# Autodesk Inventor assembly: Estructura Lámina
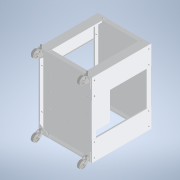
[picture p0: Inventor's stored thumbnail of the model, 180x180]
Saved by Autodesk Inventor 2021 (Build 250183000, 183)
## iProperties
Created: 2021-04-18
Part Number: Estructura Lámina
Document SubType Name: Assembly
Designer: carlo
Mass: 32488.5 g
Surface Area: 43844.9 cm^2
Volume: 4433.33 cm^3
Density: 7.32822 g/cm^3
Author: carlo
## Documents named in this file (14)
- C:\Users\Nelson\Github\Proyecto_PAI_2021\01 CAD\Estructura Lámina.iam
- C:\Users\Nelson\Github\Proyecto_PAI_2021\01 CAD\Laterales.ipt
- C:\Users\Nelson\Github\Proyecto_PAI_2021\01 CAD\Tapa.ipt
- C:\Users\Nelson\Github\Proyecto_PAI_2021\01 CAD\Ensamblaje_tapa_inferior_mesa.iam
- C:\Users\Nelson\Github\Proyecto_PAI_2021\01 CAD\Arandela_m6-din_6902-a_200hv.ipt
- C:\Users\Nelson\Github\Proyecto_PAI_2021\01 CAD\Tornillo_m6_x_l_16__iso7380-1_a2-070.ipt
- C:\Users\Nelson\Github\Proyecto_PAI_2021\01 CAD\Separador.ipt
- C:\Users\Nelson\Github\Proyecto_PAI_2021\01 CAD\Tornillo m6_x_l_12__iso7380-1_a2-070.ipt
- C:\Users\Nelson\Github\Proyecto_PAI_2021\01 CAD\Tuerca_M6_din934.ipt
- C:\Users\Nelson\Github\Proyecto_PAI_2021\01 CAD\Rueda giratoria con freno.ipt
- C:\Users\Nelson\Github\Proyecto_PAI_2021\01 CAD\Rueda giratoria.ipt
- C:\Users\Nelson\Github\Proyecto_PAI_2021\01 CAD\Grower_m10_din_6905.ipt
- C:\Users\Nelson\Github\Proyecto_PAI_2021\01 CAD\Arandela_m10-din_6902-a_200hv.ipt
- C:\Users\Nelson\Github\Proyecto_PAI_2021\01 CAD\Tornillo_m10x25-8_8_din_933.ipt
## Components (91 placed, 13 different names)
1. Tapa:1 — Coincidencia:21, Coincidencia:22, Coincidencia:23, Coincidencia:24, Coincidencia:25, Coincidencia:26, Coincidencia:27, Coincidencia:28, Coincidencia:29, Coincidencia:30, Coincidencia:31, Coincidencia:32, Mate:37
2. Laterales:1 — Coincidencia:27, Coincidencia:28, Coincidencia:29, Coincidencia:35, Mate:54, Mate:55, Mate:58, Mate:59, Mate:60, Mate:61, Mate:62, Mate:63, Mate:68, Mate:69, Mate:70, Mate:71
3. Laterales:2 — Coincidencia:21, Coincidencia:22, Coincidencia:23, Coincidencia:33, Mate:36, Mate:38, Mate:39, Mate:44, Mate:45, Mate:46, Mate:47, Mate:78, Mate:79, Mate:82, Mate:83
4. Laterales:3 — Coincidencia:24, Coincidencia:25, Coincidencia:26, Coincidencia:34, Mate:64, Mate:65, Mate:66, Mate:67, Mate:72, Mate:73, Mate:74, Mate:75, Mate:76, Mate:77, Mate:80, Mate:81
5. Laterales:4 — Coincidencia:30, Coincidencia:31, Coincidencia:32, Mate:40, Mate:41, Mate:42, Mate:43, Mate:48, Mate:49, Mate:50, Mate:51, Mate:52, Mate:53, Mate:56, Mate:57
6. Ensamblaje_tapa_inferior_mesa:1 [sub-assembly] — Coincidencia:33, Coincidencia:34, Coincidencia:35, Mate:132, Mate:133, Mate:134, Mate:135, Mate:136, Mate:137, Mate:138, Mate:139, Mate:140, Mate:160, Mate:162, Mate:164, Mate:166, Mate:168, Mate:170, Mate:172, Mate:174, Mate:176, Mate:177, Mate:178, Mate:179, Mate:180, Mate:181, Mate:182, Mate:183, Mate:184, Mate:194, Mate:196, Mate:198, Mate:200, Mate:201, Mate:203, Mate:205, Mate:207
7. Arandela_m6-din_6902-a_200hv:1 — Mate:36, Mate:37, Mate:108, Mate:109
8. Arandela_m6-din_6902-a_200hv:2 — Mate:38, Mate:39, Mate:110, Mate:111
9. Arandela_m6-din_6902-a_200hv:3 — Mate:40, Mate:41, Mate:112, Mate:113
10. Arandela_m6-din_6902-a_200hv:4 — Mate:42, Mate:43, Mate:118, Mate:119
11. Arandela_m6-din_6902-a_200hv:5 — Mate:44, Mate:45, Mate:114, Mate:115
12. Arandela_m6-din_6902-a_200hv:6 — Mate:46, Mate:47, Mate:116, Mate:117
13. Arandela_m6-din_6902-a_200hv:7 — Mate:48, Mate:49, Mate:120, Mate:121
14. Arandela_m6-din_6902-a_200hv:8 — Mate:50, Mate:51, Mate:122, Mate:123
15. Arandela_m6-din_6902-a_200hv:9 — Mate:52, Mate:53, Mate:124, Mate:125
16. Arandela_m6-din_6902-a_200hv:10 — Mate:54, Mate:55, Mate:126, Mate:127
17. Arandela_m6-din_6902-a_200hv:11 — Mate:56, Mate:57, Mate:128, Mate:129
18. Arandela_m6-din_6902-a_200hv:12 — Mate:58, Mate:59, Mate:130, Mate:131
19. Arandela_m6-din_6902-a_200hv:13 — Mate:60, Mate:61, Mate:84, Mate:85
20. Arandela_m6-din_6902-a_200hv:14 — Mate:62, Mate:63, Mate:86, Mate:87
21. Arandela_m6-din_6902-a_200hv:15 — Mate:64, Mate:65, Mate:92, Mate:93
22. Arandela_m6-din_6902-a_200hv:16 — Mate:66, Mate:67, Mate:94, Mate:95
23. Arandela_m6-din_6902-a_200hv:17 — Mate:68, Mate:69, Mate:88, Mate:89
24. Arandela_m6-din_6902-a_200hv:18 — Mate:70, Mate:71, Mate:90, Mate:91
25. Arandela_m6-din_6902-a_200hv:19 — Mate:72, Mate:73, Mate:96, Mate:97
26. Arandela_m6-din_6902-a_200hv:20 — Mate:74, Mate:75, Mate:98, Mate:99
27. Arandela_m6-din_6902-a_200hv:21 — Mate:76, Mate:77, Mate:100, Mate:101
28. Arandela_m6-din_6902-a_200hv:22 — Mate:78, Mate:79, Mate:102, Mate:103
29. Arandela_m6-din_6902-a_200hv:23 — Mate:80, Mate:81, Mate:104, Mate:105
30. Arandela_m6-din_6902-a_200hv:24 — Mate:82, Mate:83, Mate:106, Mate:107
31. Tornillo_m6_x_l_16__iso7380-1_a2-070:1 — Mate:84, Mate:85
32. Tornillo_m6_x_l_16__iso7380-1_a2-070:2 — Mate:86, Mate:87
33. Tornillo_m6_x_l_16__iso7380-1_a2-070:3 — Mate:88, Mate:89
34. Tornillo_m6_x_l_16__iso7380-1_a2-070:4 — Mate:90, Mate:91
35. Tornillo_m6_x_l_16__iso7380-1_a2-070:5 — Mate:92, Mate:93
36. Tornillo_m6_x_l_16__iso7380-1_a2-070:6 — Mate:94, Mate:95
37. Tornillo_m6_x_l_16__iso7380-1_a2-070:7 — Mate:96, Mate:97
38. Tornillo_m6_x_l_16__iso7380-1_a2-070:8 — Mate:98, Mate:99
39. Tornillo_m6_x_l_16__iso7380-1_a2-070:9 — Mate:100, Mate:101
40. Tornillo_m6_x_l_16__iso7380-1_a2-070:10 — Mate:102, Mate:103
41. Tornillo_m6_x_l_16__iso7380-1_a2-070:11 — Mate:104, Mate:105
42. Tornillo_m6_x_l_16__iso7380-1_a2-070:12 — Mate:106, Mate:107
43. Tornillo_m6_x_l_16__iso7380-1_a2-070:13 — Mate:108, Mate:109
44. Tornillo_m6_x_l_16__iso7380-1_a2-070:14 — Mate:110, Mate:111
45. Tornillo_m6_x_l_16__iso7380-1_a2-070:15 — Mate:112, Mate:113
46. Tornillo_m6_x_l_16__iso7380-1_a2-070:16 — Mate:114, Mate:115
47. Tornillo_m6_x_l_16__iso7380-1_a2-070:17 — Mate:116, Mate:117
48. Tornillo_m6_x_l_16__iso7380-1_a2-070:18 — Mate:118, Mate:119
49. Tornillo_m6_x_l_16__iso7380-1_a2-070:19 — Mate:120, Mate:121
50. Tornillo_m6_x_l_16__iso7380-1_a2-070:20 — Mate:122, Mate:123
51. Tornillo_m6_x_l_16__iso7380-1_a2-070:21 — Mate:124, Mate:125
52. Tornillo_m6_x_l_16__iso7380-1_a2-070:22 — Mate:126, Mate:127
53. Tornillo_m6_x_l_16__iso7380-1_a2-070:23 — Mate:128, Mate:129
54. Tornillo_m6_x_l_16__iso7380-1_a2-070:24 — Mate:130, Mate:131
55. Separador:1 — Mate:132, Mate:139, Mate:140, Mate:153, Mate:154, Mate:155, Mate:156, Mate:157, Mate:158
56. Separador:2 — Mate:133, Mate:137, Mate:138, Mate:147, Mate:148, Mate:149, Mate:150, Mate:151, Mate:152
57. Separador:3 — Mate:134, Mate:135, Mate:136, Mate:141, Mate:142, Mate:143, Mate:144, Mate:145, Mate:146
58. Tornillo m6_x_l_12__iso7380-1_a2-070:1 — Mate:141, Mate:142, Mate:171
59. Tornillo m6_x_l_12__iso7380-1_a2-070:2 — Mate:157, Mate:158, Mate:159
60. Tornillo m6_x_l_12__iso7380-1_a2-070:3 — Mate:153, Mate:154, Mate:163
61. Tornillo m6_x_l_12__iso7380-1_a2-070:4 — Mate:145, Mate:146, Mate:175
62. Tornillo m6_x_l_12__iso7380-1_a2-070:5 — Mate:149, Mate:150, Mate:167
63. Tornillo m6_x_l_12__iso7380-1_a2-070:6 — Mate:155, Mate:156, Mate:161
64. Tornillo m6_x_l_12__iso7380-1_a2-070:7 — Mate:143, Mate:144, Mate:173
65. Tornillo m6_x_l_12__iso7380-1_a2-070:8 — Mate:147, Mate:148, Mate:165
66. Tornillo m6_x_l_12__iso7380-1_a2-070:9 — Mate:151, Mate:152, Mate:169
67. Tuerca_M6_din934:1 — Mate:165, Mate:166
68. Tuerca_M6_din934:2 — Mate:167, Mate:168
69. Tuerca_M6_din934:3 — Mate:173, Mate:174
70. Tuerca_M6_din934:4 — Mate:169, Mate:170
71. Tuerca_M6_din934:5 — Mate:171, Mate:172
72. Tuerca_M6_din934:6 — Mate:163, Mate:164
73. Tuerca_M6_din934:7 — Mate:161, Mate:162
74. Tuerca_M6_din934:8 — Mate:175, Mate:176
75. Tuerca_M6_din934:9 — Mate:159, Mate:160
76. Rueda giratoria con freno:1 — Mate:177, Mate:179, Mate:187, Mate:188
77. Rueda giratoria con freno:2 — Mate:178, Mate:180, Mate:185, Mate:186
78. Rueda giratoria:1 — Mate:182, Mate:184, Mate:189, Mate:190
79. Rueda giratoria:2 — Mate:181, Mate:183, Mate:191, Mate:192
80. Grower_m10_din_6905:1 — Mate:185, Mate:186, Mate:193
81. Grower_m10_din_6905:2 — Mate:187, Mate:188, Mate:195
82. Grower_m10_din_6905:3 — Mate:189, Mate:190, Mate:199
83. Grower_m10_din_6905:4 — Mate:191, Mate:192, Mate:197
84. Arandela_m10-din_6902-a_200hv:1 — Mate:199, Mate:200, Mate:208
85. Arandela_m10-din_6902-a_200hv:2 — Mate:197, Mate:198, Mate:206
86. Arandela_m10-din_6902-a_200hv:3 — Mate:193, Mate:194, Mate:202
87. Arandela_m10-din_6902-a_200hv:4 — Mate:195, Mate:196, Mate:204
88. Tornillo_m10x25-8_8_din_933:1 — Mate:201, Mate:202
89. Tornillo_m10x25-8_8_din_933:2 — Mate:203, Mate:204
90. Tornillo_m10x25-8_8_din_933:3 — Mate:207, Mate:208
91. Tornillo_m10x25-8_8_din_933:4 — Mate:205, Mate:206
## Relationships (188: Mate 188)
- Coincidencia:21 [Mate]: Tapa:1 ↔ Laterales:2
- Coincidencia:22 [Mate]: Tapa:1 ↔ Laterales:2
- Coincidencia:23 [Mate]: Tapa:1 ↔ Laterales:2
- Coincidencia:24 [Mate]: Tapa:1 ↔ Laterales:3
- Coincidencia:25 [Mate]: Tapa:1 ↔ Laterales:3
- Coincidencia:26 [Mate]: Tapa:1 ↔ Laterales:3
- Coincidencia:27 [Mate]: Tapa:1 ↔ Laterales:1
- Coincidencia:28 [Mate]: Tapa:1 ↔ Laterales:1
- Coincidencia:29 [Mate]: Tapa:1 ↔ Laterales:1
- Coincidencia:30 [Mate]: Tapa:1 ↔ Laterales:4
- Coincidencia:31 [Mate]: Tapa:1 ↔ Laterales:4
- Coincidencia:32 [Mate]: Tapa:1 ↔ Laterales:4
- Coincidencia:33 [Mate]: Laterales:2 ↔ Ensamblaje_tapa_inferior_mesa:1
- Coincidencia:34 [Mate]: Laterales:3 ↔ Ensamblaje_tapa_inferior_mesa:1
- Coincidencia:35 [Mate]: Laterales:1 ↔ Ensamblaje_tapa_inferior_mesa:1
- Mate:36: Laterales:2 ↔ Arandela_m6-din_6902-a_200hv:1
- Mate:37: Tapa:1 ↔ Arandela_m6-din_6902-a_200hv:1
- Mate:38: Laterales:2 ↔ Arandela_m6-din_6902-a_200hv:2
- Mate:39: Laterales:2 ↔ Arandela_m6-din_6902-a_200hv:2
- Mate:40: Laterales:4 ↔ Arandela_m6-din_6902-a_200hv:3
- Mate:41: Laterales:4 ↔ Arandela_m6-din_6902-a_200hv:3
- Mate:42: Laterales:4 ↔ Arandela_m6-din_6902-a_200hv:4
- Mate:43: Laterales:4 ↔ Arandela_m6-din_6902-a_200hv:4
- Mate:44: Laterales:2 ↔ Arandela_m6-din_6902-a_200hv:5
- Mate:45: Laterales:2 ↔ Arandela_m6-din_6902-a_200hv:5
- Mate:46: Laterales:2 ↔ Arandela_m6-din_6902-a_200hv:6
- Mate:47: Laterales:2 ↔ Arandela_m6-din_6902-a_200hv:6
- Mate:48: Laterales:4 ↔ Arandela_m6-din_6902-a_200hv:7
- Mate:49: Laterales:4 ↔ Arandela_m6-din_6902-a_200hv:7
- Mate:50: Laterales:4 ↔ Arandela_m6-din_6902-a_200hv:8
- Mate:51: Laterales:4 ↔ Arandela_m6-din_6902-a_200hv:8
- Mate:52: Laterales:4 ↔ Arandela_m6-din_6902-a_200hv:9
- Mate:53: Laterales:4 ↔ Arandela_m6-din_6902-a_200hv:9
- Mate:54: Laterales:1 ↔ Arandela_m6-din_6902-a_200hv:10
- Mate:55: Laterales:1 ↔ Arandela_m6-din_6902-a_200hv:10
- Mate:56: Laterales:4 ↔ Arandela_m6-din_6902-a_200hv:11
- Mate:57: Laterales:4 ↔ Arandela_m6-din_6902-a_200hv:11
- Mate:58: Laterales:1 ↔ Arandela_m6-din_6902-a_200hv:12
- Mate:59: Laterales:1 ↔ Arandela_m6-din_6902-a_200hv:12
- Mate:60: Laterales:1 ↔ Arandela_m6-din_6902-a_200hv:13
- Mate:61: Laterales:1 ↔ Arandela_m6-din_6902-a_200hv:13
- Mate:62: Laterales:1 ↔ Arandela_m6-din_6902-a_200hv:14
- Mate:63: Laterales:1 ↔ Arandela_m6-din_6902-a_200hv:14
- Mate:64: Laterales:3 ↔ Arandela_m6-din_6902-a_200hv:15
- Mate:65: Laterales:3 ↔ Arandela_m6-din_6902-a_200hv:15
- Mate:66: Laterales:3 ↔ Arandela_m6-din_6902-a_200hv:16
- Mate:67: Laterales:3 ↔ Arandela_m6-din_6902-a_200hv:16
- Mate:68: Laterales:1 ↔ Arandela_m6-din_6902-a_200hv:17
- Mate:69: Laterales:1 ↔ Arandela_m6-din_6902-a_200hv:17
- Mate:70: Laterales:1 ↔ Arandela_m6-din_6902-a_200hv:18
- Mate:71: Laterales:1 ↔ Arandela_m6-din_6902-a_200hv:18
- Mate:72: Laterales:3 ↔ Arandela_m6-din_6902-a_200hv:19
- Mate:73: Laterales:3 ↔ Arandela_m6-din_6902-a_200hv:19
- Mate:74: Laterales:3 ↔ Arandela_m6-din_6902-a_200hv:20
- Mate:75: Laterales:3 ↔ Arandela_m6-din_6902-a_200hv:20
- Mate:76: Laterales:3 ↔ Arandela_m6-din_6902-a_200hv:21
- Mate:77: Laterales:3 ↔ Arandela_m6-din_6902-a_200hv:21
- Mate:78: Laterales:2 ↔ Arandela_m6-din_6902-a_200hv:22
- Mate:79: Laterales:2 ↔ Arandela_m6-din_6902-a_200hv:22
- Mate:80: Laterales:3 ↔ Arandela_m6-din_6902-a_200hv:23
- Mate:81: Laterales:3 ↔ Arandela_m6-din_6902-a_200hv:23
- Mate:82: Laterales:2 ↔ Arandela_m6-din_6902-a_200hv:24
- Mate:83: Laterales:2 ↔ Arandela_m6-din_6902-a_200hv:24
- Mate:84: Arandela_m6-din_6902-a_200hv:13 ↔ Tornillo_m6_x_l_16__iso7380-1_a2-070:1
- Mate:85: Arandela_m6-din_6902-a_200hv:13 ↔ Tornillo_m6_x_l_16__iso7380-1_a2-070:1
- Mate:86: Arandela_m6-din_6902-a_200hv:14 ↔ Tornillo_m6_x_l_16__iso7380-1_a2-070:2
- Mate:87: Arandela_m6-din_6902-a_200hv:14 ↔ Tornillo_m6_x_l_16__iso7380-1_a2-070:2
- Mate:88: Arandela_m6-din_6902-a_200hv:17 ↔ Tornillo_m6_x_l_16__iso7380-1_a2-070:3
- Mate:89: Arandela_m6-din_6902-a_200hv:17 ↔ Tornillo_m6_x_l_16__iso7380-1_a2-070:3
- Mate:90: Arandela_m6-din_6902-a_200hv:18 ↔ Tornillo_m6_x_l_16__iso7380-1_a2-070:4
- Mate:91: Arandela_m6-din_6902-a_200hv:18 ↔ Tornillo_m6_x_l_16__iso7380-1_a2-070:4
- Mate:92: Arandela_m6-din_6902-a_200hv:15 ↔ Tornillo_m6_x_l_16__iso7380-1_a2-070:5
- Mate:93: Arandela_m6-din_6902-a_200hv:15 ↔ Tornillo_m6_x_l_16__iso7380-1_a2-070:5
- Mate:94: Arandela_m6-din_6902-a_200hv:16 ↔ Tornillo_m6_x_l_16__iso7380-1_a2-070:6
- Mate:95: Arandela_m6-din_6902-a_200hv:16 ↔ Tornillo_m6_x_l_16__iso7380-1_a2-070:6
- Mate:96: Arandela_m6-din_6902-a_200hv:19 ↔ Tornillo_m6_x_l_16__iso7380-1_a2-070:7
- Mate:97: Arandela_m6-din_6902-a_200hv:19 ↔ Tornillo_m6_x_l_16__iso7380-1_a2-070:7
- Mate:98: Arandela_m6-din_6902-a_200hv:20 ↔ Tornillo_m6_x_l_16__iso7380-1_a2-070:8
- Mate:99: Arandela_m6-din_6902-a_200hv:20 ↔ Tornillo_m6_x_l_16__iso7380-1_a2-070:8
- Mate:100: Arandela_m6-din_6902-a_200hv:21 ↔ Tornillo_m6_x_l_16__iso7380-1_a2-070:9
- Mate:101: Arandela_m6-din_6902-a_200hv:21 ↔ Tornillo_m6_x_l_16__iso7380-1_a2-070:9
- Mate:102: Arandela_m6-din_6902-a_200hv:22 ↔ Tornillo_m6_x_l_16__iso7380-1_a2-070:10
- Mate:103: Arandela_m6-din_6902-a_200hv:22 ↔ Tornillo_m6_x_l_16__iso7380-1_a2-070:10
- Mate:104: Arandela_m6-din_6902-a_200hv:23 ↔ Tornillo_m6_x_l_16__iso7380-1_a2-070:11
- Mate:105: Arandela_m6-din_6902-a_200hv:23 ↔ Tornillo_m6_x_l_16__iso7380-1_a2-070:11
- Mate:106: Arandela_m6-din_6902-a_200hv:24 ↔ Tornillo_m6_x_l_16__iso7380-1_a2-070:12
- Mate:107: Arandela_m6-din_6902-a_200hv:24 ↔ Tornillo_m6_x_l_16__iso7380-1_a2-070:12
- Mate:108: Arandela_m6-din_6902-a_200hv:1 ↔ Tornillo_m6_x_l_16__iso7380-1_a2-070:13
- Mate:109: Arandela_m6-din_6902-a_200hv:1 ↔ Tornillo_m6_x_l_16__iso7380-1_a2-070:13
- Mate:110: Arandela_m6-din_6902-a_200hv:2 ↔ Tornillo_m6_x_l_16__iso7380-1_a2-070:14
- Mate:111: Arandela_m6-din_6902-a_200hv:2 ↔ Tornillo_m6_x_l_16__iso7380-1_a2-070:14
- Mate:112: Arandela_m6-din_6902-a_200hv:3 ↔ Tornillo_m6_x_l_16__iso7380-1_a2-070:15
- Mate:113: Arandela_m6-din_6902-a_200hv:3 ↔ Tornillo_m6_x_l_16__iso7380-1_a2-070:15
- Mate:114: Arandela_m6-din_6902-a_200hv:5 ↔ Tornillo_m6_x_l_16__iso7380-1_a2-070:16
- Mate:115: Arandela_m6-din_6902-a_200hv:5 ↔ Tornillo_m6_x_l_16__iso7380-1_a2-070:16
- Mate:116: Arandela_m6-din_6902-a_200hv:6 ↔ Tornillo_m6_x_l_16__iso7380-1_a2-070:17
- Mate:117: Arandela_m6-din_6902-a_200hv:6 ↔ Tornillo_m6_x_l_16__iso7380-1_a2-070:17
- Mate:118: Arandela_m6-din_6902-a_200hv:4 ↔ Tornillo_m6_x_l_16__iso7380-1_a2-070:18
- Mate:119: Arandela_m6-din_6902-a_200hv:4 ↔ Tornillo_m6_x_l_16__iso7380-1_a2-070:18
- Mate:120: Arandela_m6-din_6902-a_200hv:7 ↔ Tornillo_m6_x_l_16__iso7380-1_a2-070:19
- Mate:121: Arandela_m6-din_6902-a_200hv:7 ↔ Tornillo_m6_x_l_16__iso7380-1_a2-070:19
- Mate:122: Arandela_m6-din_6902-a_200hv:8 ↔ Tornillo_m6_x_l_16__iso7380-1_a2-070:20
- Mate:123: Arandela_m6-din_6902-a_200hv:8 ↔ Tornillo_m6_x_l_16__iso7380-1_a2-070:20
- Mate:124: Arandela_m6-din_6902-a_200hv:9 ↔ Tornillo_m6_x_l_16__iso7380-1_a2-070:21
- Mate:125: Arandela_m6-din_6902-a_200hv:9 ↔ Tornillo_m6_x_l_16__iso7380-1_a2-070:21
- Mate:126: Arandela_m6-din_6902-a_200hv:10 ↔ Tornillo_m6_x_l_16__iso7380-1_a2-070:22
- Mate:127: Arandela_m6-din_6902-a_200hv:10 ↔ Tornillo_m6_x_l_16__iso7380-1_a2-070:22
- Mate:128: Arandela_m6-din_6902-a_200hv:11 ↔ Tornillo_m6_x_l_16__iso7380-1_a2-070:23
- Mate:129: Arandela_m6-din_6902-a_200hv:11 ↔ Tornillo_m6_x_l_16__iso7380-1_a2-070:23
- Mate:130: Arandela_m6-din_6902-a_200hv:12 ↔ Tornillo_m6_x_l_16__iso7380-1_a2-070:24
- Mate:131: Arandela_m6-din_6902-a_200hv:12 ↔ Tornillo_m6_x_l_16__iso7380-1_a2-070:24
- Mate:132: Ensamblaje_tapa_inferior_mesa:1 ↔ Separador:1
- Mate:133: Ensamblaje_tapa_inferior_mesa:1 ↔ Separador:2
- Mate:134: Ensamblaje_tapa_inferior_mesa:1 ↔ Separador:3
- Mate:135: Ensamblaje_tapa_inferior_mesa:1 ↔ Separador:3
- Mate:136: Ensamblaje_tapa_inferior_mesa:1 ↔ Separador:3
- Mate:137: Ensamblaje_tapa_inferior_mesa:1 ↔ Separador:2
- Mate:138: Ensamblaje_tapa_inferior_mesa:1 ↔ Separador:2
- Mate:139: Ensamblaje_tapa_inferior_mesa:1 ↔ Separador:1
- Mate:140: Ensamblaje_tapa_inferior_mesa:1 ↔ Separador:1
- Mate:141: Separador:3 ↔ Tornillo m6_x_l_12__iso7380-1_a2-070:1
- Mate:142: Separador:3 ↔ Tornillo m6_x_l_12__iso7380-1_a2-070:1
- Mate:143: Separador:3 ↔ Tornillo m6_x_l_12__iso7380-1_a2-070:7
- Mate:144: Separador:3 ↔ Tornillo m6_x_l_12__iso7380-1_a2-070:7
- Mate:145: Separador:3 ↔ Tornillo m6_x_l_12__iso7380-1_a2-070:4
- Mate:146: Separador:3 ↔ Tornillo m6_x_l_12__iso7380-1_a2-070:4
- Mate:147: Separador:2 ↔ Tornillo m6_x_l_12__iso7380-1_a2-070:8
- Mate:148: Separador:2 ↔ Tornillo m6_x_l_12__iso7380-1_a2-070:8
- Mate:149: Separador:2 ↔ Tornillo m6_x_l_12__iso7380-1_a2-070:5
- Mate:150: Separador:2 ↔ Tornillo m6_x_l_12__iso7380-1_a2-070:5
- Mate:151: Separador:2 ↔ Tornillo m6_x_l_12__iso7380-1_a2-070:9
- Mate:152: Separador:2 ↔ Tornillo m6_x_l_12__iso7380-1_a2-070:9
- Mate:153: Separador:1 ↔ Tornillo m6_x_l_12__iso7380-1_a2-070:3
- Mate:154: Separador:1 ↔ Tornillo m6_x_l_12__iso7380-1_a2-070:3
- Mate:155: Separador:1 ↔ Tornillo m6_x_l_12__iso7380-1_a2-070:6
- Mate:156: Separador:1 ↔ Tornillo m6_x_l_12__iso7380-1_a2-070:6
- Mate:157: Separador:1 ↔ Tornillo m6_x_l_12__iso7380-1_a2-070:2
- Mate:158: Separador:1 ↔ Tornillo m6_x_l_12__iso7380-1_a2-070:2
- Mate:159: Tornillo m6_x_l_12__iso7380-1_a2-070:2 ↔ Tuerca_M6_din934:9
- Mate:160: Ensamblaje_tapa_inferior_mesa:1 ↔ Tuerca_M6_din934:9
- Mate:161: Tornillo m6_x_l_12__iso7380-1_a2-070:6 ↔ Tuerca_M6_din934:7
- Mate:162: Ensamblaje_tapa_inferior_mesa:1 ↔ Tuerca_M6_din934:7
- Mate:163: Tornillo m6_x_l_12__iso7380-1_a2-070:3 ↔ Tuerca_M6_din934:6
- Mate:164: Ensamblaje_tapa_inferior_mesa:1 ↔ Tuerca_M6_din934:6
- Mate:165: Tornillo m6_x_l_12__iso7380-1_a2-070:8 ↔ Tuerca_M6_din934:1
- Mate:166: Ensamblaje_tapa_inferior_mesa:1 ↔ Tuerca_M6_din934:1
- Mate:167: Tornillo m6_x_l_12__iso7380-1_a2-070:5 ↔ Tuerca_M6_din934:2
- Mate:168: Ensamblaje_tapa_inferior_mesa:1 ↔ Tuerca_M6_din934:2
- Mate:169: Tornillo m6_x_l_12__iso7380-1_a2-070:9 ↔ Tuerca_M6_din934:4
- Mate:170: Ensamblaje_tapa_inferior_mesa:1 ↔ Tuerca_M6_din934:4
- Mate:171: Tornillo m6_x_l_12__iso7380-1_a2-070:1 ↔ Tuerca_M6_din934:5
- Mate:172: Ensamblaje_tapa_inferior_mesa:1 ↔ Tuerca_M6_din934:5
- Mate:173: Tornillo m6_x_l_12__iso7380-1_a2-070:7 ↔ Tuerca_M6_din934:3
- Mate:174: Ensamblaje_tapa_inferior_mesa:1 ↔ Tuerca_M6_din934:3
- Mate:175: Tornillo m6_x_l_12__iso7380-1_a2-070:4 ↔ Tuerca_M6_din934:8
- Mate:176: Ensamblaje_tapa_inferior_mesa:1 ↔ Tuerca_M6_din934:8
- Mate:177: Ensamblaje_tapa_inferior_mesa:1 ↔ Rueda giratoria con freno:1
- Mate:178: Ensamblaje_tapa_inferior_mesa:1 ↔ Rueda giratoria con freno:2
- Mate:179: Ensamblaje_tapa_inferior_mesa:1 ↔ Rueda giratoria con freno:1
- Mate:180: Ensamblaje_tapa_inferior_mesa:1 ↔ Rueda giratoria con freno:2
- Mate:181: Ensamblaje_tapa_inferior_mesa:1 ↔ Rueda giratoria:2
- Mate:182: Ensamblaje_tapa_inferior_mesa:1 ↔ Rueda giratoria:1
- Mate:183: Ensamblaje_tapa_inferior_mesa:1 ↔ Rueda giratoria:2
- Mate:184: Ensamblaje_tapa_inferior_mesa:1 ↔ Rueda giratoria:1
- Mate:185: Rueda giratoria con freno:2 ↔ Grower_m10_din_6905:1
- Mate:186: Rueda giratoria con freno:2 ↔ Grower_m10_din_6905:1
- Mate:187: Rueda giratoria con freno:1 ↔ Grower_m10_din_6905:2
- Mate:188: Rueda giratoria con freno:1 ↔ Grower_m10_din_6905:2
- Mate:189: Rueda giratoria:1 ↔ Grower_m10_din_6905:3
- Mate:190: Rueda giratoria:1 ↔ Grower_m10_din_6905:3
- Mate:191: Rueda giratoria:2 ↔ Grower_m10_din_6905:4
- Mate:192: Rueda giratoria:2 ↔ Grower_m10_din_6905:4
- Mate:193: Grower_m10_din_6905:1 ↔ Arandela_m10-din_6902-a_200hv:3
- Mate:194: Ensamblaje_tapa_inferior_mesa:1 ↔ Arandela_m10-din_6902-a_200hv:3
- Mate:195: Grower_m10_din_6905:2 ↔ Arandela_m10-din_6902-a_200hv:4
- Mate:196: Ensamblaje_tapa_inferior_mesa:1 ↔ Arandela_m10-din_6902-a_200hv:4
- Mate:197: Grower_m10_din_6905:4 ↔ Arandela_m10-din_6902-a_200hv:2
- Mate:198: Ensamblaje_tapa_inferior_mesa:1 ↔ Arandela_m10-din_6902-a_200hv:2
- Mate:199: Grower_m10_din_6905:3 ↔ Arandela_m10-din_6902-a_200hv:1
- Mate:200: Ensamblaje_tapa_inferior_mesa:1 ↔ Arandela_m10-din_6902-a_200hv:1
- Mate:201: Ensamblaje_tapa_inferior_mesa:1 ↔ Tornillo_m10x25-8_8_din_933:1
- Mate:202: Arandela_m10-din_6902-a_200hv:3 ↔ Tornillo_m10x25-8_8_din_933:1
- Mate:203: Ensamblaje_tapa_inferior_mesa:1 ↔ Tornillo_m10x25-8_8_din_933:2
- Mate:204: Arandela_m10-din_6902-a_200hv:4 ↔ Tornillo_m10x25-8_8_din_933:2
- Mate:205: Ensamblaje_tapa_inferior_mesa:1 ↔ Tornillo_m10x25-8_8_din_933:4
- Mate:206: Arandela_m10-din_6902-a_200hv:2 ↔ Tornillo_m10x25-8_8_din_933:4
- Mate:207: Ensamblaje_tapa_inferior_mesa:1 ↔ Tornillo_m10x25-8_8_din_933:3
- Mate:208: Arandela_m10-din_6902-a_200hv:1 ↔ Tornillo_m10x25-8_8_din_933:3
## Named parameters: sa_0 = 0, sa_1 = -981, sa_2 = 0
note: some values were not read from the file. Shown as the stored number, unit unknown: "sa_0", "sa_1", "sa_2".
